# Autodesk Inventor assembly: Assembly1
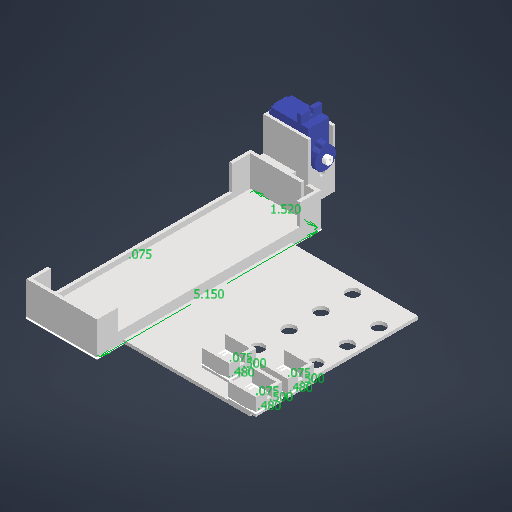
[picture p0: Inventor's stored thumbnail of the model, 512x512]
Saved by Autodesk Inventor 2026.2 (Build 302298010, 298A)
## iProperties
Created: 2026-03-08
Part Number: Assembly1
Document SubType Name: Assembly
Designer: david
Author: david
## Documents named in this file (4)
- C:\Users\david\Documents\UIUC\ECE 445\Assembly1.iam
- C:\Users\david\Documents\UIUC\ECE 445\HarmonicaFrame.ipt
- C:\Users\david\Documents\UIUC\ECE 445\SG90_Model_A.ipt
- C:\Users\david\Documents\UIUC\ECE 445\SolenoidHolder.ipt
## Components (5 placed, 3 different names)
1. HarmonicaFrame:1 — Insert:1, Insert:2, Insert:3, Insert:4
2. SG90_Model_A:1 — Insert:1
3. SolenoidHolder:1 — Insert:2
4. SolenoidHolder:2 — Insert:4
5. SolenoidHolder:3 — Insert:3
## Relationships (4: Insert 4)
- Insert:1: HarmonicaFrame:1 ↔ SG90_Model_A:1
- Insert:2: HarmonicaFrame:1 ↔ SolenoidHolder:1
- Insert:3: HarmonicaFrame:1 ↔ SolenoidHolder:3
- Insert:4: HarmonicaFrame:1 ↔ SolenoidHolder:2
